# Autodesk Inventor assembly: LidAssem
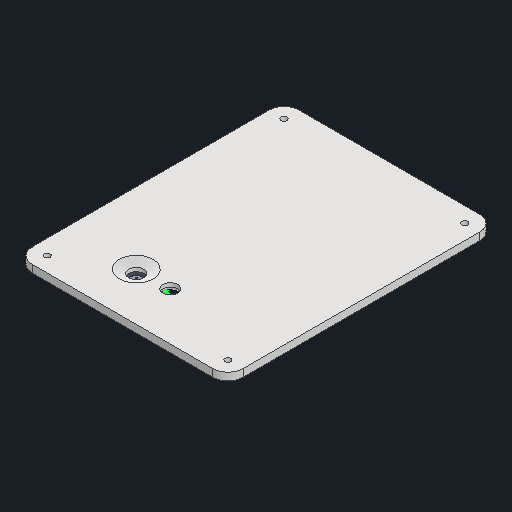
[picture p0: Inventor's stored thumbnail of the model, 512x512]
Saved by Autodesk Inventor 2026.2 (Build 302298000, 298)
## iProperties
Created: 2026-02-21
Part Number: LidAssem
Document SubType Name: Assembly
Designer: niuke
Author: niuke
## Documents named in this file (3)
- C:\Users\niuke\Documents\GitHub\angel-box\CAD\LidAssem.iam
- C:\Users\niuke\Documents\GitHub\angel-box\CAD\Parts\Logitech C270\C270.ipt
- C:\Users\niuke\Documents\GitHub\angel-box\CAD\Lid.ipt
## Components (2 placed, 2 different names)
1. C270:1 — Flush:1, Flush:2
2. Lid:1 — Flush:1, Flush:2
## Relationships (2: Flush 2)
- Flush:1: C270:1 ↔ Lid:1
- Flush:2 (10.9982 mm): C270:1 ↔ Lid:1
